# Autodesk Inventor assembly: locomotionsubsytem2
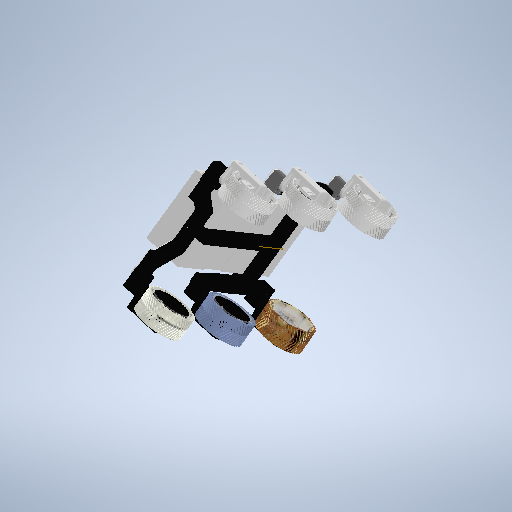
[picture p0: Inventor's stored thumbnail of the model, 512x512]
Saved by Autodesk Inventor 2025.3 (Build 293356000, 356)
## iProperties
Created: 2026-04-18
Part Number: locomotionsubsytem2
Document SubType Name: Assembly
Designer: ksawe
Author: ksawe
## Documents named in this file (6)
- C:\Users\ksawe\OneDrive\Pulpit\Exomy v1\wersja3\locomotionsubsytem2.iam
- C:\Users\ksawe\OneDrive\Pulpit\Exomy v1\wersja3\pairofwheels.iam
- C:\Users\ksawe\OneDrive\Pulpit\Exomy v1\wersja3\wheelbasketback.iam
- C:\Users\ksawe\OneDrive\Pulpit\Exomy v1\wersja3\T.iam
- C:\Users\ksawe\OneDrive\Pulpit\Exomy v1\wersja3\handler_back.ipt
- C:\Users\ksawe\OneDrive\Pulpit\Exomy v1\wersja3\nakladka_back.ipt
## Components (7 placed, 5 different names)
1. pairofwheels:1 [sub-assembly] — Rotational:4
2. pairofwheels:2 [sub-assembly] — Rotational:6
3. wheelbasketback:1 [sub-assembly] — Mate:13, Mate:14, Mate:15
4. wheelbasketback:2 [sub-assembly] — Mate:10, Mate:11, Mate:16
5. T:1 [sub-assembly] — Rotational:4, Rotational:5, Rotational:6
6. handler_back:1 — Rotational:5, Mate:7, Mate:9, Mate:10, Mate:11, Mate:13, Mate:14, Mate:15, Mate:16, Mate:17
7. nakladka_back:1 — Mate:7, Mate:9, Mate:17
## Relationships (12: Mate 9, RevoluteJoint 3)
- Rotational:4 [RevoluteJoint]: pairofwheels:1 ↔ T:1
- Rotational:5 [RevoluteJoint]: T:1 ↔ handler_back:1
- Rotational:6 [RevoluteJoint]: pairofwheels:2 ↔ T:1
- Mate:7: handler_back:1 ↔ nakladka_back:1
- Mate:9: handler_back:1 ↔ nakladka_back:1
- Mate:10: wheelbasketback:2 ↔ handler_back:1
- Mate:11: wheelbasketback:2 ↔ handler_back:1
- Mate:13: wheelbasketback:1 ↔ handler_back:1
- Mate:14: wheelbasketback:1 ↔ handler_back:1
- Mate:15: wheelbasketback:1 ↔ handler_back:1
- Mate:16: wheelbasketback:2 ↔ handler_back:1
- Mate:17: handler_back:1 ↔ nakladka_back:1
